# Autodesk Inventor assembly: Track_pad
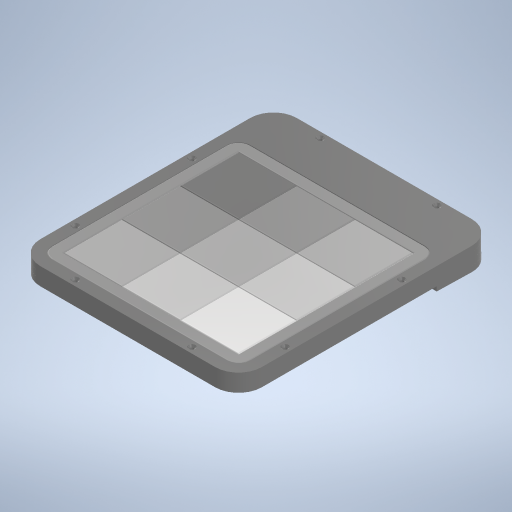
[picture p0: Inventor's stored thumbnail of the model, 512x512]
Saved by Autodesk Inventor 2023 (Build 270158000, 158)
## iProperties
Created: 2022-11-05
Part Number: Track_pad
Document SubType Name: Assembly
Designer: RubenStein
Mass: 610.347 g
Surface Area: 2886.57 cm^2
Volume: 610.347 cm^3
Density: 1 g/cm^3
Author: RubenStein
## Documents named in this file (7)
- C:\Users\RubenStein\OneDrive - mci4me.at\Documents\Track_Pad\Track_pad.iam
- C:\Users\RubenStein\OneDrive - mci4me.at\Documents\Track_Pad\Plate_mount.ipt
- C:\Users\RubenStein\OneDrive - mci4me.at\Documents\Track_Pad\frame_outer.ipt
- C:\Users\RubenStein\OneDrive - mci4me.at\Documents\Track_Pad\frame_inner.ipt
- C:\Users\RubenStein\OneDrive - mci4me.at\Documents\Track_Pad\Tile.ipt
- C:\Users\RubenStein\OneDrive - mci4me.at\Documents\Track_Pad\Plate_bottom.ipt
- C:\Users\RubenStein\OneDrive - mci4me.at\Documents\Track_Pad\foot.ipt
## Components (14 placed, 6 different names)
1. Plate_mount:1 — Passend:1, Fluchtend:1, Fluchtend:2, Passend:4, Fluchtend:16, Fluchtend:17, Passend:19
2. frame_outer:1 — Passend:1, Fluchtend:1, Fluchtend:2, Passend:2, Passend:3
3. frame_inner:1 — Passend:2, Passend:3, Passend:4, Passend:17, Passend:18, Fluchtend:15
4. Tile:1 — Passend:9, Fluchtend:8, Fluchtend:9, Passend:10
5. Tile:2 — Passend:6, Fluchtend:4, Fluchtend:6, Passend:7, Fluchtend:7, Passend:9, Fluchtend:8, Fluchtend:9
6. Tile:3 — Passend:5, Fluchtend:3, Passend:6, Fluchtend:4, Fluchtend:5, Fluchtend:6, Fluchtend:15
7. Tile:4 — Passend:5, Fluchtend:3, Fluchtend:5, Passend:8, Passend:12, Fluchtend:11, Fluchtend:12
8. Tile:5 — Passend:7, Passend:8, Fluchtend:7, Passend:11, Fluchtend:10, Passend:13
9. Tile:6 — Passend:12, Fluchtend:11, Fluchtend:12, Passend:14, Fluchtend:13, Passend:17, Passend:18
10. Tile:7 — Passend:13, Passend:14, Fluchtend:13, Passend:16, Fluchtend:14
11. Tile:8 — Passend:15, Passend:16, Fluchtend:14
12. Tile:9 — Passend:10, Passend:11, Fluchtend:10, Passend:15
13. Plate_bottom:1 — Fluchtend:16, Fluchtend:17, Passend:19, Fluchtend:18, Fluchtend:19, Passend:20
14. foot:1 — Fluchtend:18, Fluchtend:19, Passend:20
## Relationships (39: Mate 20, Flush 19)
- Passend:1 [Mate]: Plate_mount:1 ↔ frame_outer:1
- Fluchtend:1 [Flush]: Plate_mount:1 ↔ frame_outer:1
- Fluchtend:2 [Flush]: Plate_mount:1 ↔ frame_outer:1
- Passend:2 [Mate]: frame_outer:1 ↔ frame_inner:1
- Passend:3 [Mate]: frame_outer:1 ↔ frame_inner:1
- Passend:4 [Mate]: Plate_mount:1 ↔ frame_inner:1
- Passend:5 [Mate]: Tile:3 ↔ Tile:4
- Fluchtend:3 [Flush]: Tile:3 ↔ Tile:4
- Passend:6 [Mate]: Tile:2 ↔ Tile:3
- Fluchtend:4 [Flush]: Tile:2 ↔ Tile:3
- Fluchtend:5 [Flush]: Tile:3 ↔ Tile:4
- Fluchtend:6 [Flush]: Tile:2 ↔ Tile:3
- Passend:7 [Mate]: Tile:2 ↔ Tile:5
- Passend:8 [Mate]: Tile:4 ↔ Tile:5
- Fluchtend:7 [Flush]: Tile:2 ↔ Tile:5
- Passend:9 [Mate]: Tile:1 ↔ Tile:2
- Fluchtend:8 [Flush]: Tile:1 ↔ Tile:2
- Fluchtend:9 [Flush]: Tile:1 ↔ Tile:2
- Passend:10 [Mate]: Tile:1 ↔ Tile:9
- Passend:11 [Mate]: Tile:5 ↔ Tile:9
- Fluchtend:10 [Flush]: Tile:5 ↔ Tile:9
- Passend:12 [Mate]: Tile:4 ↔ Tile:6
- Fluchtend:11 [Flush]: Tile:4 ↔ Tile:6
- Fluchtend:12 [Flush]: Tile:4 ↔ Tile:6
- Passend:13 [Mate]: Tile:5 ↔ Tile:7
- Passend:14 [Mate]: Tile:6 ↔ Tile:7
- Fluchtend:13 [Flush]: Tile:6 ↔ Tile:7
- Passend:15 [Mate]: Tile:8 ↔ Tile:9
- Passend:16 [Mate]: Tile:7 ↔ Tile:8
- Fluchtend:14 [Flush]: Tile:7 ↔ Tile:8
- Passend:17 [Mate]: frame_inner:1 ↔ Tile:6
- Passend:18 [Mate]: frame_inner:1 ↔ Tile:6
- Fluchtend:15 [Flush]: frame_inner:1 ↔ Tile:3
- Fluchtend:16 [Flush]: Plate_mount:1 ↔ Plate_bottom:1
- Fluchtend:17 [Flush]: Plate_mount:1 ↔ Plate_bottom:1
- Passend:19 [Mate]: Plate_mount:1 ↔ Plate_bottom:1
- Fluchtend:18 [Flush]: Plate_bottom:1 ↔ foot:1
- Fluchtend:19 [Flush]: Plate_bottom:1 ↔ foot:1
- Passend:20 [Mate]: Plate_bottom:1 ↔ foot:1
